# Autodesk Inventor assembly: CNC-X-axis- ASSEMBLY
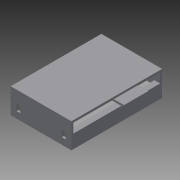
[picture p0: Inventor's stored thumbnail of the model, 180x180]
Saved by Autodesk Inventor 2015 (Build 190159000, 159)
## iProperties
Created: 2015-03-24
Part Number: CNC-X-axis- ASSEMBLY
Document SubType Name: Assembly
Designer: Bangladesh
Author: Bangladesh
## Documents named in this file (11)
- C:\Users\Alvi\Documents\CNC design files\Assemblies\CNC-X-axis- ASSEMBLY.iam
- C:\Users\Alvi\Documents\CNC design files\CNC-X-axis- main 2 by 4.ipt
- C:\Users\Alvi\Documents\CNC design files\CNC-X-axis- linear drawer slider.ipt
- C:\Users\Alvi\Documents\CNC design files\CNC-X-axis- front plate drawer exits.ipt
- C:\Users\Alvi\Documents\CNC design files\CNC-X-axis- drawer block.ipt
- C:\Users\Alvi\Documents\CNC design files\CNC-X-axis- platform mover.ipt
- C:\Users\Alvi\Documents\CNC design files\CNC-X-axis- foundation faces.ipt
- C:\Users\Alvi\Documents\CNC design files\CNC- Stepper Motor.ipt
- C:\Users\Alvi\Documents\CNC design files\CNC-X-axis- moving platform.ipt
- C:\Users\Alvi\Documents\CNC design files\CNC- Hexagonal Bit.ipt
- C:\Users\Alvi\Documents\CNC design files\CNC-X-axis- bed platform.ipt
## Components (13 placed, 10 different names)
1. CNC-X-axis- main 2 by 4:1 — Mate:7, Mate:8, Mate:9, Mate:31, Mate:32, Mate:39
2. CNC-X-axis- main 2 by 4:2 — Mate:10, Mate:11, Mate:12, Mate:38
3. CNC-X-axis- linear drawer slider:1 — Mate:7, Mate:8, Mate:9, Mate:13, Mate:14, Mate:19, Mate:20, Mate:21, Mate:22
4. CNC-X-axis- linear drawer slider:2 — Mate:10, Mate:11, Mate:12, Mate:15, Mate:16, Mate:17, Mate:18, Mate:25
5. CNC-X-axis- drawer block:1 — Mate:13, Mate:14, Mate:19, Mate:20, Mate:21, Mate:22, Mate:36, Mate:37, Mate:41
6. CNC-X-axis- drawer block:2 — Mate:15, Mate:16, Mate:17, Mate:18, Mate:25, Mate:40
7. CNC-X-axis- foundation faces:1 — Mate:31, Mate:32, Mate:34, Mate:35, Mate:44
8. CNC- Stepper Motor:1 — Mate:34, Mate:35
9. CNC-X-axis- platform mover:1 — Mate:36, Mate:37, Mate:42, Mate:43
10. CNC-X-axis- front plate drawer exits:1 — Mate:38, Mate:39, Mate:45
11. CNC-X-axis- moving platform:1 — Mate:40, Mate:41
12. CNC- Hexagonal Bit:1 — Mate:42, Mate:43
13. CNC-X-axis- bed platform:1 — Mate:44, Mate:45
## Relationships (31: Mate 31)
- Mate:7: CNC-X-axis- main 2 by 4:1 ↔ CNC-X-axis- linear drawer slider:1
- Mate:8: CNC-X-axis- main 2 by 4:1 ↔ CNC-X-axis- linear drawer slider:1
- Mate:9 (43.18 mm): CNC-X-axis- main 2 by 4:1 ↔ CNC-X-axis- linear drawer slider:1
- Mate:10: CNC-X-axis- main 2 by 4:2 ↔ CNC-X-axis- linear drawer slider:2
- Mate:11: CNC-X-axis- main 2 by 4:2 ↔ CNC-X-axis- linear drawer slider:2
- Mate:12 (43.18 mm): CNC-X-axis- main 2 by 4:2 ↔ CNC-X-axis- linear drawer slider:2
- Mate:13: CNC-X-axis- linear drawer slider:1 ↔ CNC-X-axis- drawer block:1
- Mate:14: CNC-X-axis- linear drawer slider:1 ↔ CNC-X-axis- drawer block:1
- Mate:15: CNC-X-axis- linear drawer slider:2 ↔ CNC-X-axis- drawer block:2
- Mate:16: CNC-X-axis- linear drawer slider:2 ↔ CNC-X-axis- drawer block:2
- Mate:17: CNC-X-axis- linear drawer slider:2 ↔ CNC-X-axis- drawer block:2
- Mate:18 (334.348 mm): CNC-X-axis- linear drawer slider:2 ↔ CNC-X-axis- drawer block:2
- Mate:19: CNC-X-axis- linear drawer slider:1 ↔ CNC-X-axis- drawer block:1
- Mate:20: CNC-X-axis- linear drawer slider:1 ↔ CNC-X-axis- drawer block:1
- Mate:21: CNC-X-axis- linear drawer slider:1 ↔ CNC-X-axis- drawer block:1
- Mate:22 (334.348 mm): CNC-X-axis- linear drawer slider:1 ↔ CNC-X-axis- drawer block:1
- Mate:25: CNC-X-axis- linear drawer slider:2 ↔ CNC-X-axis- drawer block:2
- Mate:31: CNC-X-axis- main 2 by 4:1 ↔ CNC-X-axis- foundation faces:1
- Mate:32: CNC-X-axis- main 2 by 4:1 ↔ CNC-X-axis- foundation faces:1
- Mate:34: CNC-X-axis- foundation faces:1 ↔ CNC- Stepper Motor:1
- Mate:35: CNC-X-axis- foundation faces:1 ↔ CNC- Stepper Motor:1
- Mate:36: CNC-X-axis- drawer block:1 ↔ CNC-X-axis- platform mover:1
- Mate:37: CNC-X-axis- drawer block:1 ↔ CNC-X-axis- platform mover:1
- Mate:38: CNC-X-axis- main 2 by 4:2 ↔ CNC-X-axis- front plate drawer exits:1
- Mate:39: CNC-X-axis- main 2 by 4:1 ↔ CNC-X-axis- front plate drawer exits:1
- Mate:40: CNC-X-axis- drawer block:2 ↔ CNC-X-axis- moving platform:1
- Mate:41 (-93.5 mm): CNC-X-axis- drawer block:1 ↔ CNC-X-axis- moving platform:1
- Mate:42: CNC-X-axis- platform mover:1 ↔ CNC- Hexagonal Bit:1
- Mate:43: CNC-X-axis- platform mover:1 ↔ CNC- Hexagonal Bit:1
- Mate:44: CNC-X-axis- foundation faces:1 ↔ CNC-X-axis- bed platform:1
- Mate:45: CNC-X-axis- front plate drawer exits:1 ↔ CNC-X-axis- bed platform:1
